# Autodesk Inventor assembly: bilmiyorum
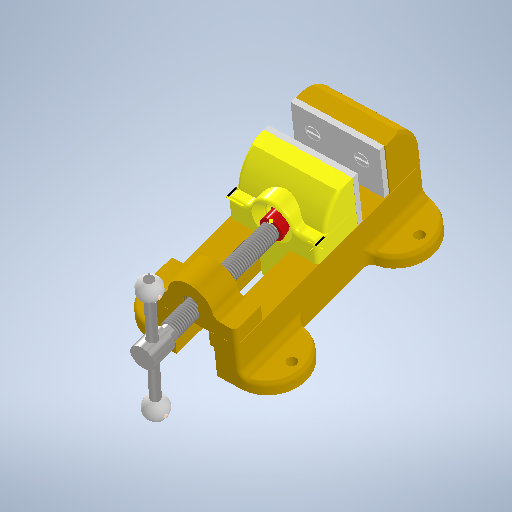
[picture p0: Inventor's stored thumbnail of the model, 512x512]
Saved by Autodesk Inventor 2025.4 (Build 294407000, 407)
## iProperties
Created: 2026-06-22
Part Number: bilmiyorum
Document SubType Name: Assembly
Designer: win10
Author: win10
## Documents named in this file (3)
- C:\Users\win10\Desktop\cad-final-projesi\bilmiyorum.iam
- C:\Users\win10\Desktop\cad-final-projesi\VİDA_MİLİ2.iam
- C:\Users\win10\Desktop\cad-final-projesi\vidasız montaj.iam
## Components (2 placed, 2 different names)
1. VİDA_MİLİ2:1 [sub-assembly] — Mate:1
2. vidasız montaj:1 [sub-assembly] — Mate:1
## Relationships (1: Mate 1)
- Mate:1: VİDA_MİLİ2:1 ↔ vidasız montaj:1
